# Autodesk Inventor assembly: Assembly_box_kit
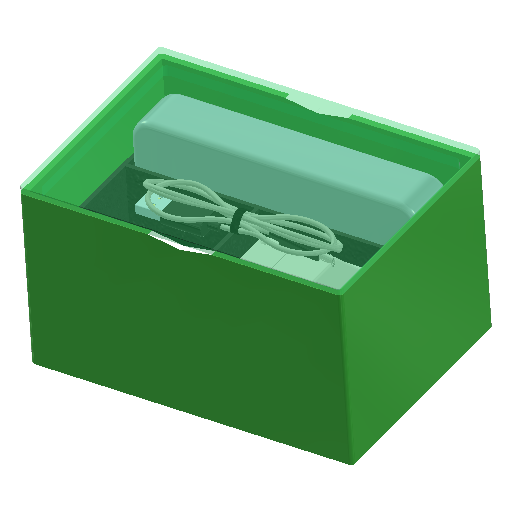
[picture p0: Inventor's stored thumbnail of the model, 512x512]
Saved by Autodesk Inventor 2026.1 (Build 301233020, 233B)
## iProperties
Created: 2026-02-19
Part Number: Assembly_box_kit
Document SubType Name: Assembly
Designer: samuel
Author: samuel
## Documents named in this file (10)
- E:\Fraunhofer\Design\Assembly_box_kit.iam
- E:\Fraunhofer\Design\Assembly_Box.iam
- E:\Fraunhofer\Design\Parts\powerbank.ipt
- E:\Fraunhofer\Design\box_kit.ipt
- E:\Fraunhofer\Design\Parts\ads1015 ads1115 module type1\ads1015 ads1115 module type1\ads1015 ads1115 module type1.ipt
- E:\Fraunhofer\Design\Parts\Beetle ESP32-C6\Beetle ESP32-C6\Beetle ESP32-C6.ipt
- E:\Fraunhofer\Design\Assembly_NV_Module.iam
- E:\Fraunhofer\Design\Assembly_Optical_Module.iam
- E:\Fraunhofer\Design\Parts\coiled USB cable\coiled USB cable\coiled USB cable.ipt
- E:\Fraunhofer\Design\box_kit_lid.ipt
## Components (9 placed, 9 different names)
1. Assembly_Box:1 [sub-assembly] — Mate:5, Mate:6, Mate:9
2. powerbank:1 — Mate:2, Mate:3, Mate:8
3. box_kit:1 — Mate:2, Mate:3, Mate:5, Mate:6, Mate:8, Mate:9, Mate:10, Mate:12, Mate:13, Mate:14, Mate:15, Mate:16, Mate:17, Mate:18, Flush:1, Flush:2
4. ads1015 ads1115 module type1:1 — Mate:10
5. Beetle ESP32-C6:1 — Mate:15, Mate:16
6. Assembly_NV_Module:1 [sub-assembly] — Mate:13, Mate:17
7. Assembly_Optical_Module:1 [sub-assembly] — Mate:12, Mate:14
8. coiled USB cable:1 — Mate:18
9. box_kit_lid:1 — Flush:1, Flush:2
## Relationships (16: Mate 14, Flush 2)
- Mate:2 (1 mm): powerbank:1 ↔ box_kit:1
- Mate:3 (1 mm): powerbank:1 ↔ box_kit:1
- Mate:5 (1 mm): Assembly_Box:1 ↔ box_kit:1
- Mate:6 (1 mm): Assembly_Box:1 ↔ box_kit:1
- Mate:8: powerbank:1 ↔ box_kit:1
- Mate:9: Assembly_Box:1 ↔ box_kit:1
- Mate:10 (7 mm): box_kit:1 ↔ ads1015 ads1115 module type1:1
- Mate:12: box_kit:1 ↔ Assembly_Optical_Module:1
- Mate:13: box_kit:1 ↔ Assembly_NV_Module:1
- Mate:14: box_kit:1 ↔ Assembly_Optical_Module:1
- Mate:15: box_kit:1 ↔ Beetle ESP32-C6:1
- Mate:16: box_kit:1 ↔ Beetle ESP32-C6:1
- Mate:17: box_kit:1 ↔ Assembly_NV_Module:1
- Mate:18 (30 mm): box_kit:1 ↔ coiled USB cable:1
- Flush:1: box_kit:1 ↔ box_kit_lid:1
- Flush:2: box_kit:1 ↔ box_kit_lid:1
